# Autodesk Inventor assembly: Motor Modul
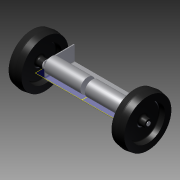
[picture p0: Inventor's stored thumbnail of the model, 180x180]
Saved by Autodesk Inventor 2014 (Build 180170000, 170)
## iProperties
Created: 2014-02-18
Part Number: Motor Modul
Document SubType Name: Assembly
Designer: Pinkponk
Author: Pinkponk
## Documents named in this file (5)
- X:\Projekt\Min Robot\Min Robot\Motor Modul.iam
- X:\Projekt\Min Robot\Min Robot\Hjul.ipt
- X:\Projekt\Min Robot\Min Robot\Hjul Motor.ipt
- X:\Projekt\Min Robot\Min Robot\Hjulstopp.ipt
- X:\Projekt\Min Robot\Min Robot\MotorPlatta.ipt
## Components (7 placed, 4 different names)
1. Hjul:1 — Insert:1
2. Hjul:2 — Insert:2
3. Hjul Motor:1 — Insert:4, Angle:1, Insert:5
4. Hjul Motor:2 — Insert:3, Angle:2, Insert:6
5. Hjulstopp:1 — Insert:2, Insert:4
6. Hjulstopp:2 — Insert:1, Insert:3
7. MotorPlatta:1 — Angle:1, Insert:5, Angle:2, Insert:6
## Relationships (8: Insert 6, Angle 2)
- Insert:1: Hjul:1 ↔ Hjulstopp:2
- Insert:2: Hjul:2 ↔ Hjulstopp:1
- Insert:3: Hjul Motor:2 ↔ Hjulstopp:2
- Insert:4: Hjul Motor:1 ↔ Hjulstopp:1
- Angle:1 (180 deg): Hjul Motor:1 ↔ MotorPlatta:1
- Insert:5: Hjul Motor:1 ↔ MotorPlatta:1
- Angle:2 (180 deg): Hjul Motor:2 ↔ MotorPlatta:1
- Insert:6: Hjul Motor:2 ↔ MotorPlatta:1
